# Autodesk Inventor assembly: LargeGearInput
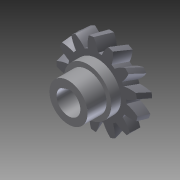
[picture p0: Inventor's stored thumbnail of the model, 180x180]
Saved by Autodesk Inventor 2012 (Build 160160000, 160)
## iProperties
Created: 2011-10-26
Part Number: LargeGearInput
Document SubType Name: Assembly
Designer: akutta
Author: akutta
## Documents named in this file (3)
- C:\Users\KuttaA\Dropbox\Hexapod Research\Leg Design\Other Parts\Intermediary Gear Box\Assemblies\LargeGearInput.iam
- C:\Users\KuttaA\Dropbox\Hexapod Research\Leg Design\Other Parts\Intermediary Gear Box\gear\Design Accelerator\Spur Gear21.ipt
- C:\Users\KuttaA\Dropbox\Hexapod Research\Leg Design\Other Parts\Intermediary Gear Box\Assemblies\BlankLargeGearMotorInput.ipt
## Components (2 placed, 2 different names)
1. Spur Gear2:1 — Mate:1, Mate:2
2. BlankLargeGearMotorInput:1 — Mate:1, Mate:2
## Relationships (2: Mate 2)
- Mate:1: Spur Gear2:1 ↔ BlankLargeGearMotorInput:1
- Mate:2: Spur Gear2:1 ↔ BlankLargeGearMotorInput:1
